# Autodesk Inventor assembly: 4 Flex, HS
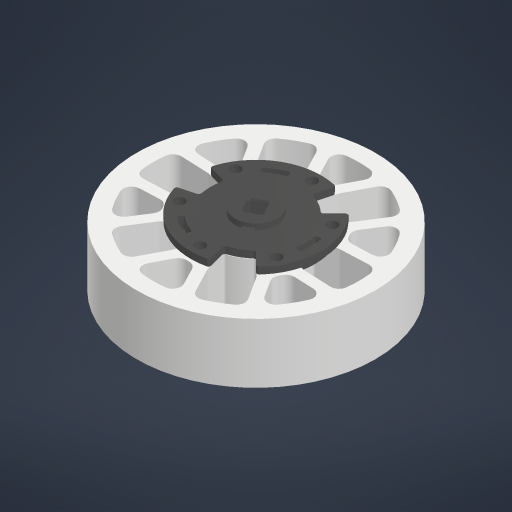
[picture p0: Inventor's stored thumbnail of the model, 512x512]
Saved by Autodesk Inventor 2023 (Build 270158000, 158)
## iProperties
Created: 2023-02-19
Part Number: 4 Flex, HS
Document SubType Name: Assembly
Designer: Windows Macbook
Author: Windows Macbook
## Documents named in this file (5)
- C:\Users\Windows Macbook\Desktop\Inventor\Motion\Wheels\Flex Wheels\4 Flex, HS.iam
- C:\Users\Windows Macbook\Desktop\Inventor\Motion\Wheels\Flex Wheels\4.000 Flex Wheel\4.000 30A 1.000.ipt
- C:\Users\Windows Macbook\Desktop\Inventor\Motion\Wheels\Flex Wheels\4.000 Flex Wheel.ipt
- C:\Users\Windows Macbook\Desktop\Inventor\Motion\Wheels\Flex Wheels\VersaHub.ipt
- C:\Users\Windows Macbook\Desktop\Inventor\Motion\Wheels\Flex Wheels\VersaHex Adapters .250.ipt
## Components (5 placed, 3 different names)
1. 4.000 30A 1.000:1 — Insert:5, Insert:6, Insert:7, Insert:8
2. VersaHub:2 — Insert:3, Mate:1, Insert:5, Insert:6
3. VersaHex Adapters .250:1 — Insert:3, Mate:1
4. VersaHub:3 — Insert:7, Insert:8, Mate:2
5. VersaHex Adapters .250:3 — Mate:2
## Relationships (8: Insert 6, Mate 2)
- Insert:3: VersaHub:2 ↔ VersaHex Adapters .250:1
- Mate:1: VersaHub:2 ↔ VersaHex Adapters .250:1
- [Insert]: VersaHub:3 ↔ VersaHex Adapters .250:3
- Insert:5: 4.000 30A 1.000:1 ↔ VersaHub:2
- Insert:6: 4.000 30A 1.000:1 ↔ VersaHub:2
- Insert:7: 4.000 30A 1.000:1 ↔ VersaHub:3
- Insert:8: 4.000 30A 1.000:1 ↔ VersaHub:3
- Mate:2: VersaHub:3 ↔ VersaHex Adapters .250:3
## Named parameters: d6_d3 = 0 mm
